# Autodesk Inventor assembly: MainAssembly
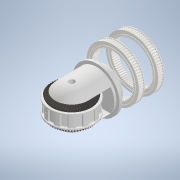
[picture p0: Inventor's stored thumbnail of the model, 180x180]
Saved by Autodesk Inventor 2020 (Build 240168000, 168)
## iProperties
Created: 2019-05-09
Part Number: MainAssembly
Document SubType Name: Assembly
Designer: Connor
Author: Connor
## Documents named in this file (6)
- C:\Users\Connor\Documents\GrabCAD\DifferentialSwerve\MainAssembly.iam
- C:\Users\Connor\Documents\GrabCAD\DifferentialSwerve\RingGearAssembly.iam
- C:\Users\Connor\Documents\GrabCAD\DifferentialSwerve\Imported Components\Wheels and Hubs\VEX Traction Wheels\TractionWheel 4x1\TractionWheel 4x1.iam
- C:\Users\Connor\Documents\GrabCAD\DifferentialSwerve\15t_bevel.ipt
- C:\Users\Connor\Documents\GrabCAD\DifferentialSwerve\60t_bevel.ipt
- C:\Users\Connor\Documents\GrabCAD\DifferentialSwerve\PlanetaryFrame.ipt
## Components (8 placed, 5 different names)
1. RingGearAssembly:1 [sub-assembly] — Mate:10
2. TractionWheel 4x1:1 [sub-assembly] — Mate:1, Mate:2, Mate:3, Mate:4, Mate:5, Mate:6, Mate:11
3. 15t_bevel:1 — Tangent:1, Flush:1, Mate:7
4. 60t_bevel:1 — Mate:4, Mate:5, Mate:6, Tangent:1, Flush:1, Mate:7
5. 15t_bevel:2 — Tangent:2, Mate:9, Flush:2
6. 60t_bevel:2 — Mate:1, Mate:2, Mate:3, Tangent:2, Mate:9, Flush:2
7. RingGearAssembly:2 [sub-assembly] — Mate:10
8. PlanetaryFrame:1 — Mate:11
## Relationships (14: Mate 10, Tangent 2, Flush 2)
- Mate:1: TractionWheel 4x1:1 ↔ 60t_bevel:2
- Mate:2: TractionWheel 4x1:1 ↔ 60t_bevel:2
- Mate:3: TractionWheel 4x1:1 ↔ 60t_bevel:2
- Mate:4: TractionWheel 4x1:1 ↔ 60t_bevel:1
- Mate:5: TractionWheel 4x1:1 ↔ 60t_bevel:1
- Mate:6: TractionWheel 4x1:1 ↔ 60t_bevel:1
- Tangent:1 (2 mm): 15t_bevel:1 ↔ 60t_bevel:1
- Flush:1 (56 mm): 15t_bevel:1 ↔ 60t_bevel:1
- Mate:7: 15t_bevel:1 ↔ 60t_bevel:1
- Tangent:2 (2 mm): 15t_bevel:2 ↔ 60t_bevel:2
- Mate:9 (-56 mm): 15t_bevel:2 ↔ 60t_bevel:2
- Flush:2: 15t_bevel:2 ↔ 60t_bevel:2
- Mate:10: RingGearAssembly:1 ↔ RingGearAssembly:2
- Mate:11: TractionWheel 4x1:1 ↔ PlanetaryFrame:1
